# Autodesk Inventor assembly: Rb PEEK_Rb PEEK - Abajo_PZ
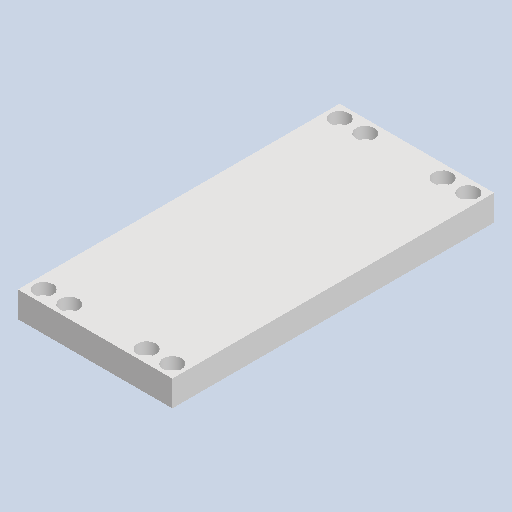
[picture p0: Inventor's stored thumbnail of the model, 512x512]
Saved by Autodesk Inventor 2025.3 (Build 293356000, 356)
## iProperties
Created: 2025-05-09
Part Number: Rb PEEK_Rb PEEK - Abajo_PZ
Document SubType Name: Assembly
Designer: Verðandi
Author: Verðandi
## Documents named in this file (2)
- E:\Users\USER\Documents\GitHub\LAFriOC\Rb oven housing\Rb oven housing\Rb PEEK_Rb PEEK - Abajo_PZ.iam
- E:\Users\USER\Documents\GitHub\LAFriOC\Rb oven housing\Rb oven housing\Rb PEEK_Rb PEEK - Abajo_MP.ipt
## Components (1 placed, 1 different names)
1. Rb PEEK_Rb PEEK - Abajo_MP:1 — Flush:1, Flush:2, Flush:3
## Relationships (3: Flush 3)
- Flush:1: Rb PEEK_Rb PEEK - Abajo_MP:1
- Flush:2: Rb PEEK_Rb PEEK - Abajo_MP:1
- Flush:3: Rb PEEK_Rb PEEK - Abajo_MP:1
